# Autodesk Inventor assembly: SingleSiCMonofilamentPrintHead
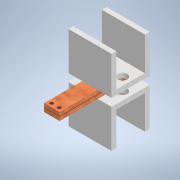
[picture p0: Inventor's stored thumbnail of the model, 180x180]
Saved by Autodesk Inventor 2021 (Build 250183000, 183)
## iProperties
Created: 2021-12-02
Part Number: SingleSiCMonofilamentPrintHead
Document SubType Name: Assembly
Designer: Unit-005
Author: Unit-005
## Documents named in this file (6)
- C:\Users\Unit-005\Documents\Inventor\SiC_Monofilament_MicroheaterPrinthead\SingleSiCMonofilamentPrintHead.iam
- C:\Users\Unit-005\Documents\Inventor\SiC_Monofilament_MicroheaterPrinthead\SiCMonofilamentShort.ipt
- C:\Users\Unit-005\Documents\Inventor\SiC_Monofilament_MicroheaterPrinthead\Leads+ChannelForSingleHeater.ipt
- C:\Users\Unit-005\Documents\Inventor\SiC_Monofilament_MicroheaterPrinthead\halfinchCChannel.ipt
- C:\Users\Unit-005\Documents\Inventor\SiC_Monofilament_MicroheaterPrinthead\Leads+ChannelForSingleHeater_MIR1.ipt
- C:\Users\Unit-005\Documents\Inventor\SiC_Monofilament_MicroheaterPrinthead\halfinchCChannel_MIR.ipt
## Components (5 placed, 5 different names)
1. SiCMonofilamentShort:1 — Mate:1, Tangent:1, Mate:3, Mate:4
2. Leads+ChannelForSingleHeater:1 — Mate:1, Tangent:1, Mate:2, Flush:2, Mate:3
3. halfinchCChannel:1 — Mate:2, Flush:2, Mate:4
4. Leads+ChannelForSingleHeater_MIR1:1 — Flush:3, Mate:5
5. halfinchCChannel_MIR:1 — Flush:3, Mate:5
## Relationships (8: Mate 5, Flush 2, Tangent 1)
- Mate:1 (-0.0635 mm): SiCMonofilamentShort:1 ↔ Leads+ChannelForSingleHeater:1
- Tangent:1: SiCMonofilamentShort:1 ↔ Leads+ChannelForSingleHeater:1
- Mate:2: Leads+ChannelForSingleHeater:1 ↔ halfinchCChannel:1
- Flush:2: Leads+ChannelForSingleHeater:1 ↔ halfinchCChannel:1
- Mate:3: SiCMonofilamentShort:1 ↔ Leads+ChannelForSingleHeater:1
- Mate:4: SiCMonofilamentShort:1 ↔ halfinchCChannel:1
- Flush:3: Leads+ChannelForSingleHeater_MIR1:1 ↔ halfinchCChannel_MIR:1
- Mate:5: Leads+ChannelForSingleHeater_MIR1:1 ↔ halfinchCChannel_MIR:1
